# Autodesk Inventor assembly: Overall_Assembly_Rev3
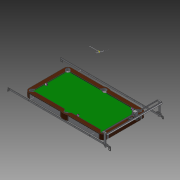
[picture p0: Inventor's stored thumbnail of the model, 180x180]
Saved by Autodesk Inventor 2015 (Build 190159000, 159)
## iProperties
Created: 2017-01-22
Part Number: Overall_Assembly_Rev3
Document SubType Name: Assembly
Designer: Guy
Author: Guy
## Documents named in this file (11)
- C:\Users\Guy\Documents\Fourth Year\Capstone\git\Capstone-Project\doc\CAD\LowLevel_Rev3\Overall_Assembly_Rev3.iam
- C:\Users\Guy\Documents\Fourth Year\Capstone\git\Capstone-Project\doc\CAD\Pool Table\Table_Model.ipt
- C:\Users\Guy\Documents\Fourth Year\Capstone\git\Capstone-Project\doc\CAD\LowLevel_Rev3\X_rail_Assembly_Rev3.iam
- C:\Users\Guy\Documents\Fourth Year\Capstone\git\Capstone-Project\doc\CAD\LowLevel_Rev3\Y_rail_Assembly_Rev3.iam
- C:\Users\Guy\Documents\Fourth Year\Capstone\git\Capstone-Project\doc\CAD\LowLevel_Rev3\Piston_Model.ipt
- C:\Users\Guy\Documents\Fourth Year\Capstone\git\Capstone-Project\doc\CAD\LowLevel_Rev2\Pool_Ball_Stripe.ipt
- C:\Users\Guy\Documents\Fourth Year\Capstone\git\Capstone-Project\doc\CAD\Nuts and Bolts\1-2in_13tpi x 8 in.ipt
- C:\Users\Guy\Documents\Fourth Year\Capstone\git\Capstone-Project\doc\CAD\ShootingMechanism\ShootingMechanism.iam
- C:\Users\Guy\Documents\Fourth Year\Capstone\git\Capstone-Project\doc\CAD\Nuts and Bolts\3-16in_1 1-4in_Bolt.ipt
- C:\Users\Guy\Documents\Fourth Year\Capstone\git\Capstone-Project\doc\CAD\Nuts and Bolts\3-16in_7-16in_washer(num8).ipt
- C:\Users\Guy\Documents\Fourth Year\Capstone\git\Capstone-Project\doc\CAD\Nuts and Bolts\3-16in_1-16in_nut(num2).ipt
## Components (21 placed, 10 different names)
1. Table_Model:1 — Tangent:1, Tangent:2, Tangent:3, Tangent:4, Tangent:5, Tangent:6, Mate:49, Mate:52, Mate:57, Mate:58, Mate:63, Mate:64
2. Pool_Ball_Stripe:1 — Tangent:1, Tangent:2
3. Pool_Ball_Stripe:2 — Tangent:3, Tangent:4
4. Pool_Ball_Stripe:3 — Tangent:5, Tangent:6
5. 1-2in_13tpi x 8 in:1 — Mate:55, Mate:56, Mate:57
6. 1-2in_13tpi x 8 in:2 — Mate:53, Mate:54, Mate:58
7. 1-2in_13tpi x 8 in:3 — Mate:49, Mate:60, Mate:62
8. 1-2in_13tpi x 8 in:4 — Mate:52, Mate:59, Mate:61
9. X_rail_Assembly_Rev3:1 [sub-assembly] — Mate:53, Mate:54, Mate:55, Mate:56, Mate:64, Flush:1, Mate:65, Mate:66, Mate:70, Mate:72, Mate:74, Mate:76, Mate:85, Mate:86
10. X_rail_Assembly_Rev3:2 [sub-assembly] — Mate:59, Mate:60, Mate:61, Mate:62, Mate:63, Flush:1, Mate:67
11. Y_rail_Assembly_Rev3:1 [sub-assembly] — Mate:65, Mate:66, Mate:67, Mate:68, Flush:2
12. Piston_Model:1
13. ShootingMechanism:1 [sub-assembly] — Mate:68, Flush:2
14. 3-16in_1 1-4in_Bolt:1 — Mate:70, Mate:75, Mate:77, Mate:84
15. 3-16in_1 1-4in_Bolt:2 — Mate:72, Mate:73, Mate:78, Mate:83
16. 3-16in_7-16in_washer(num8):1 — Mate:73, Mate:74, Mate:78
17. 3-16in_7-16in_washer(num8):2 — Mate:75, Mate:76, Mate:77
18. 3-16in_7-16in_washer(num8):3 — Mate:79, Mate:82, Mate:86
19. 3-16in_7-16in_washer(num8):4 — Mate:80, Mate:81, Mate:85
20. 3-16in_1-16in_nut(num2):1 — Mate:80, Mate:81, Mate:84
21. 3-16in_1-16in_nut(num2):2 — Mate:79, Mate:82, Mate:83
## Relationships (42: Mate 34, Tangent 6, Flush 2)
- Tangent:1: Table_Model:1 ↔ Pool_Ball_Stripe:1
- Tangent:2: Table_Model:1 ↔ Pool_Ball_Stripe:1
- Tangent:3: Table_Model:1 ↔ Pool_Ball_Stripe:2
- Tangent:4: Table_Model:1 ↔ Pool_Ball_Stripe:2
- Tangent:5: Table_Model:1 ↔ Pool_Ball_Stripe:3
- Tangent:6: Table_Model:1 ↔ Pool_Ball_Stripe:3
- Mate:49: Table_Model:1 ↔ 1-2in_13tpi x 8 in:3
- Mate:52: Table_Model:1 ↔ 1-2in_13tpi x 8 in:4
- Mate:53: 1-2in_13tpi x 8 in:2 ↔ X_rail_Assembly_Rev3:1
- Mate:54: 1-2in_13tpi x 8 in:2 ↔ X_rail_Assembly_Rev3:1
- Mate:55: 1-2in_13tpi x 8 in:1 ↔ X_rail_Assembly_Rev3:1
- Mate:56: 1-2in_13tpi x 8 in:1 ↔ X_rail_Assembly_Rev3:1
- Mate:57: Table_Model:1 ↔ 1-2in_13tpi x 8 in:1
- Mate:58: Table_Model:1 ↔ 1-2in_13tpi x 8 in:2
- Mate:59: 1-2in_13tpi x 8 in:4 ↔ X_rail_Assembly_Rev3:2
- Mate:60: 1-2in_13tpi x 8 in:3 ↔ X_rail_Assembly_Rev3:2
- Mate:61: 1-2in_13tpi x 8 in:4 ↔ X_rail_Assembly_Rev3:2
- Mate:62: 1-2in_13tpi x 8 in:3 ↔ X_rail_Assembly_Rev3:2
- Mate:63 (130 mm): Table_Model:1 ↔ X_rail_Assembly_Rev3:2
- Mate:64 (130 mm): Table_Model:1 ↔ X_rail_Assembly_Rev3:1
- Flush:1: X_rail_Assembly_Rev3:1 ↔ X_rail_Assembly_Rev3:2
- Mate:65: X_rail_Assembly_Rev3:1 ↔ Y_rail_Assembly_Rev3:1
- Mate:66: X_rail_Assembly_Rev3:1 ↔ Y_rail_Assembly_Rev3:1
- Mate:67: X_rail_Assembly_Rev3:2 ↔ Y_rail_Assembly_Rev3:1
- Mate:68: Y_rail_Assembly_Rev3:1 ↔ ShootingMechanism:1
- Flush:2: Y_rail_Assembly_Rev3:1 ↔ ShootingMechanism:1
- Mate:70: X_rail_Assembly_Rev3:1 ↔ 3-16in_1 1-4in_Bolt:1
- Mate:72: X_rail_Assembly_Rev3:1 ↔ 3-16in_1 1-4in_Bolt:2
- Mate:73: 3-16in_1 1-4in_Bolt:2 ↔ 3-16in_7-16in_washer(num8):1
- Mate:74: X_rail_Assembly_Rev3:1 ↔ 3-16in_7-16in_washer(num8):1
- Mate:75: 3-16in_1 1-4in_Bolt:1 ↔ 3-16in_7-16in_washer(num8):2
- Mate:76: X_rail_Assembly_Rev3:1 ↔ 3-16in_7-16in_washer(num8):2
- Mate:77: 3-16in_1 1-4in_Bolt:1 ↔ 3-16in_7-16in_washer(num8):2
- Mate:78: 3-16in_1 1-4in_Bolt:2 ↔ 3-16in_7-16in_washer(num8):1
- Mate:79: 3-16in_7-16in_washer(num8):3 ↔ 3-16in_1-16in_nut(num2):2
- Mate:80: 3-16in_7-16in_washer(num8):4 ↔ 3-16in_1-16in_nut(num2):1
- Mate:81: 3-16in_7-16in_washer(num8):4 ↔ 3-16in_1-16in_nut(num2):1
- Mate:82: 3-16in_7-16in_washer(num8):3 ↔ 3-16in_1-16in_nut(num2):2
- Mate:83: 3-16in_1 1-4in_Bolt:2 ↔ 3-16in_1-16in_nut(num2):2
- Mate:84: 3-16in_1 1-4in_Bolt:1 ↔ 3-16in_1-16in_nut(num2):1
- Mate:85: X_rail_Assembly_Rev3:1 ↔ 3-16in_7-16in_washer(num8):4
- Mate:86: X_rail_Assembly_Rev3:1 ↔ 3-16in_7-16in_washer(num8):3
